# Autodesk Inventor assembly: xtion_internal
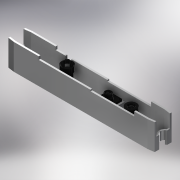
[picture p0: Inventor's stored thumbnail of the model, 180x180]
Saved by Autodesk Inventor 2017 (Build 210142000, 142)
## iProperties
Created: 2016-11-18
Part Number: xtion_internal
Document SubType Name: Assembly
Designer: Ali
Author: Ali
## Documents named in this file (5)
- C:\Users\Ali\Dropbox\Work\HeadSLAM\xtion_internal.iam
- C:\Users\Ali\Dropbox\Work\HeadSLAM\xtion_heatsink.ipt
- C:\Users\Ali\Dropbox\Work\HeadSLAM\xtion_projector.ipt
- C:\Users\Ali\Dropbox\Work\HeadSLAM\xtion_rgb_cam.ipt
- C:\Users\Ali\Dropbox\Work\HeadSLAM\xtion_ir_cam.ipt
## Components (4 placed, 4 different names)
1. xtion_heatsink:1 — Rigid:1, Rigid:2, Rigid:3
2. xtion_projector:1 — Rigid:1
3. xtion_rgb_cam:1 — Rigid:2
4. xtion_ir_cam:1 — Rigid:3
## Relationships (3: WeldJoint 3)
- Rigid:1 [WeldJoint]: xtion_heatsink:1 ↔ xtion_projector:1
- Rigid:2 [WeldJoint]: xtion_heatsink:1 ↔ xtion_rgb_cam:1
- Rigid:3 [WeldJoint]: xtion_heatsink:1 ↔ xtion_ir_cam:1
